# Autodesk Inventor assembly: Assembly1
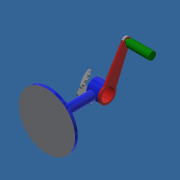
[picture p0: Inventor's stored thumbnail of the model, 180x180]
Saved by Autodesk Inventor 2018 (Build 220112000, 112)
## iProperties
Created: 2022-02-21
Part Number: Assembly1
Document SubType Name: Assembly
Designer: Nathann
Author: Nathann
## Documents named in this file (6)
- C:\Users\Nathann\OneDrive\Objet3D\EPFLEplucheCarrote\Assembly1.iam
- C:\Users\Nathann\OneDrive\Objet3D\EPFLEplucheCarrote\Feet.ipt
- C:\Users\Nathann\OneDrive\Objet3D\EPFLEplucheCarrote\Manivelle.ipt
- C:\Users\Nathann\OneDrive\Objet3D\EPFLEplucheCarrote\Handle.ipt
- C:\Users\Nathann\OneDrive\Objet3D\EPFLEplucheCarrote\Blade.ipt
- C:\Users\Nathann\OneDrive\Objet3D\EPFLEplucheCarrote\CarotGear.ipt
## Components (6 placed, 5 different names)
1. Feet:1 — Flush:1, Insert:1
2. Manivelle:1 — Flush:1, Flush:2, Insert:1
3. Handle:1 — Flush:2
4. Blade:1
5. CarotGear:1
6. CarotGear:2
## Relationships (3: Flush 2, Insert 1)
- Flush:1: Feet:1 ↔ Manivelle:1
- Flush:2: Manivelle:1 ↔ Handle:1
- Insert:1: Feet:1 ↔ Manivelle:1
